# Autodesk Inventor assembly: Intake Prototypes
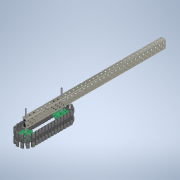
[picture p0: Inventor's stored thumbnail of the model, 180x180]
Saved by Autodesk Inventor 2020 (Build 240168000, 168)
## iProperties
Created: 2019-09-15
Part Number: Intake Prototypes
Document SubType Name: Assembly
Designer: Corey
Author: Corey
## Documents named in this file (7)
- C:\Users\Corey\Documents\Tower-Takeover-CAD\Intake Prototypes.iam
- C:\Users\Corey\Documents\Tower-Takeover-CAD\Parts\Structure\C-Channels\Aluminum\2-Wide\Aluminum C-Channel 1x2x1x35.ipt
- C:\Users\Corey\Documents\Tower-Takeover-CAD\Parts\Motion\Sprockets\High Strength 12-tooth Sprocket.ipt
- C:\Users\Corey\Documents\Tower-Takeover-CAD\Parts\Motion\Chain & Tank Tread\Tank Tread Traction Link.ipt
- C:\Users\Corey\Documents\Tower-Takeover-CAD\Parts\Motion\Bearing Flat.ipt
- C:\Users\Corey\Documents\Tower-Takeover-CAD\Chain Sketch for Intake.ipt
- C:\Users\Corey\Documents\Tower-Takeover-CAD\Parts\Motion\Drive Shafts\Drive Shaft 4''.ipt
## Components (45 placed, 6 different names)
1. Aluminum C-Channel 1x2x1x35:2 — Mate:1, Insert:1, Insert:2, Mate:2, Insert:3, Insert:4, Mate:3, Mate:4, Insert:5, Insert:6, Insert:7, Insert:8, Mate:10, Mate:17, Mate:18
2. High Strength 12-tooth Sprocket:1 — Mate:5, Mate:6, Mate:17
3. High Strength 12-tooth Sprocket:2 — Mate:7, Mate:8, Mate:18
4. Bearing Flat:1 — Mate:1, Insert:1, Insert:2
5. Bearing Flat:2 — Mate:3, Insert:5, Insert:6, Insert:9
6. Bearing Flat:3 — Mate:2, Insert:3, Insert:4
7. Bearing Flat:5 — Mate:4, Insert:7, Insert:8, Insert:10
8. Chain Sketch for Intake:1 — Mate:10, Mate:11, Mate:12, Mate:13, Mate:15, Flush:1, Mate:16
9. Drive Shaft 4'':1 — Insert:10, Mate:7, Mate:8, Mate:13
10. Drive Shaft 4'':2 — Insert:9, Mate:5, Mate:6, Mate:11, Mate:12
11. Tank Tread Traction Link:1 — Mate:15, Flush:1, Mate:16
12. Tank Tread Traction Link:2
13. Tank Tread Traction Link:3
14. Tank Tread Traction Link:4
15. Tank Tread Traction Link:5
16. Tank Tread Traction Link:6
17. Tank Tread Traction Link:7
18. Tank Tread Traction Link:8
19. Tank Tread Traction Link:9
20. Tank Tread Traction Link:10
21. Tank Tread Traction Link:11
22. Tank Tread Traction Link:12
23. Tank Tread Traction Link:13
24. Tank Tread Traction Link:14
25. Tank Tread Traction Link:15
26. Tank Tread Traction Link:16
27. Tank Tread Traction Link:17
28. Tank Tread Traction Link:18
29. Tank Tread Traction Link:19
30. Tank Tread Traction Link:20
31. Tank Tread Traction Link:21
32. Tank Tread Traction Link:22
33. Tank Tread Traction Link:23
34. Tank Tread Traction Link:24
35. Tank Tread Traction Link:25
36. Tank Tread Traction Link:26
37. Tank Tread Traction Link:27
38. Tank Tread Traction Link:28
39. Tank Tread Traction Link:29
40. Tank Tread Traction Link:30
41. Tank Tread Traction Link:31
42. Tank Tread Traction Link:32
43. Tank Tread Traction Link:33
44. Tank Tread Traction Link:34
45. Tank Tread Traction Link:35
## Component patterns: (35 elements, first: Tank Tread Traction Link:1)
## Relationships (27: Mate 16, Insert 10, Flush 1)
- Mate:1: Aluminum C-Channel 1x2x1x35:2 ↔ Bearing Flat:1
- Insert:1: Aluminum C-Channel 1x2x1x35:2 ↔ Bearing Flat:1
- Insert:2: Aluminum C-Channel 1x2x1x35:2 ↔ Bearing Flat:1
- Mate:2: Aluminum C-Channel 1x2x1x35:2 ↔ Bearing Flat:3
- Insert:3: Aluminum C-Channel 1x2x1x35:2 ↔ Bearing Flat:3
- Insert:4: Aluminum C-Channel 1x2x1x35:2 ↔ Bearing Flat:3
- Mate:3: Aluminum C-Channel 1x2x1x35:2 ↔ Bearing Flat:2
- Mate:4: Aluminum C-Channel 1x2x1x35:2 ↔ Bearing Flat:5
- Insert:5: Aluminum C-Channel 1x2x1x35:2 ↔ Bearing Flat:2
- Insert:6: Aluminum C-Channel 1x2x1x35:2 ↔ Bearing Flat:2
- Insert:7: Aluminum C-Channel 1x2x1x35:2 ↔ Bearing Flat:5
- Insert:8: Aluminum C-Channel 1x2x1x35:2 ↔ Bearing Flat:5
- Insert:9 (-25.4 mm): Bearing Flat:2 ↔ Drive Shaft 4'':2
- Insert:10 (-25.4 mm): Bearing Flat:5 ↔ Drive Shaft 4'':1
- Mate:5: High Strength 12-tooth Sprocket:1 ↔ Drive Shaft 4'':2
- Mate:6: High Strength 12-tooth Sprocket:1 ↔ Drive Shaft 4'':2
- Mate:7: High Strength 12-tooth Sprocket:2 ↔ Drive Shaft 4'':1
- Mate:8: High Strength 12-tooth Sprocket:2 ↔ Drive Shaft 4'':1
- Mate:10 (22.86 mm): Aluminum C-Channel 1x2x1x35:2 ↔ Chain Sketch for Intake:1
- Mate:11: Chain Sketch for Intake:1 ↔ Drive Shaft 4'':2
- Mate:12: Chain Sketch for Intake:1 ↔ Drive Shaft 4'':2
- Mate:13: Chain Sketch for Intake:1 ↔ Drive Shaft 4'':1
- Mate:15: Chain Sketch for Intake:1 ↔ Tank Tread Traction Link:1
- Flush:1 (24.13 mm): Chain Sketch for Intake:1 ↔ Tank Tread Traction Link:1
- Mate:16 (114.3 mm): Chain Sketch for Intake:1 ↔ Tank Tread Traction Link:1
- Mate:17 (15.24 mm): Aluminum C-Channel 1x2x1x35:2 ↔ High Strength 12-tooth Sprocket:1
- Mate:18 (15.24 mm): Aluminum C-Channel 1x2x1x35:2 ↔ High Strength 12-tooth Sprocket:2
